# Autodesk Inventor assembly: Base_Sos
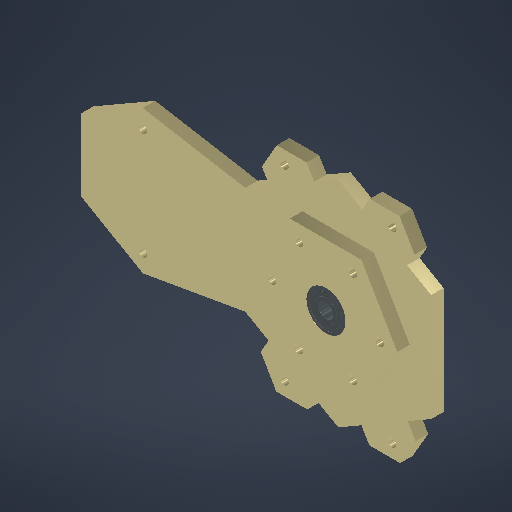
[picture p0: Inventor's stored thumbnail of the model, 512x512]
Saved by Autodesk Inventor 2025.3 (Build 293356000, 356)
## iProperties
Created: 2025-04-18
Part Number: Base_Sos
Document SubType Name: Assembly
Designer: Nelson
Author: Nelson
## Documents named in this file (3)
- C:\Users\Nelson\Documents\Inventor\SCARA\Base_Sos.iam
- C:\Users\Nelson\Documents\Inventor\SCARA\Base_STABLE.ipt
- C:\Users\Nelson\Documents\Inventor\SCARA\skf_bearing_608-2z_2.iam
## Components (2 placed, 2 different names)
1. Base_STABLE:1 — Mate:1, Mate:2, Mate:3
2. skf_bearing_608-2z_2:1 [sub-assembly] — Mate:2, Mate:3
## Relationships (3: Mate 3)
- Mate:1: Base_STABLE:1
- Mate:2: Base_STABLE:1 ↔ skf_bearing_608-2z_2:1
- Mate:3: Base_STABLE:1 ↔ skf_bearing_608-2z_2:1
